# Autodesk Inventor assembly: minutes
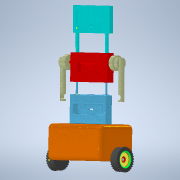
[picture p0: Inventor's stored thumbnail of the model, 180x180]
Saved by Autodesk Inventor 2021.3 (Build 253353000, 353)
## iProperties
Created: 2021-07-10
Part Number: minutes
Document SubType Name: Assembly
Designer: HP
Author: HP
## Documents named in this file (8)
- D:\exploration\final model\minutes.iam
- D:\exploration\final model\middle part edited.ipt
- D:\exploration\final model\part3nn.ipt
- D:\exploration\final model\upper part edited.ipt
- D:\exploration\final model\Partslst.ipt
- D:\exploration\final model\bottom box.ipt
- D:\exploration\final model\axel 180mm.ipt
- D:\exploration\final model\wheel 2.ipt
## Components (9 placed, 7 different names)
1. middle part edited:1 — Mate:1, Mate:2, Mate:3, Mate:4, Mate:5, Mate:6
2. part3nn:1 — Mate:1, Mate:2, Rigid:1
3. upper part edited:1 — Mate:3, Mate:4
4. Partslst:5 — Mate:5
5. Partslst:6 — Mate:6
6. bottom box:1 — Rigid:1, Mate:7, Mate:9, Mate:11
7. axel 180mm:1 — Mate:7, Mate:8, Mate:10
8. wheel 2:1 — Mate:8, Mate:9
9. wheel 2:2 — Mate:10, Mate:11
## Relationships (12: Mate 11, WeldJoint 1)
- Mate:1: middle part edited:1 ↔ part3nn:1
- Mate:2: middle part edited:1 ↔ part3nn:1
- Mate:3: middle part edited:1 ↔ upper part edited:1
- Mate:4: middle part edited:1 ↔ upper part edited:1
- Mate:5: middle part edited:1 ↔ Partslst:5
- Mate:6: middle part edited:1 ↔ Partslst:6
- Rigid:1 [WeldJoint]: part3nn:1 ↔ bottom box:1
- Mate:7: bottom box:1 ↔ axel 180mm:1
- Mate:8: axel 180mm:1 ↔ wheel 2:1
- Mate:9 (2 mm): bottom box:1 ↔ wheel 2:1
- Mate:10: axel 180mm:1 ↔ wheel 2:2
- Mate:11 (2 mm): bottom box:1 ↔ wheel 2:2
